# Autodesk Inventor assembly: сборка пульта
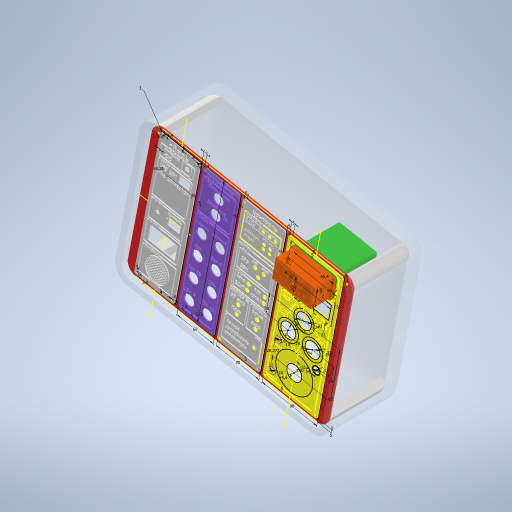
[picture p0: Inventor's stored thumbnail of the model, 512x512]
Saved by Autodesk Inventor 2023.2 (Build 272271000, 271)
## iProperties
Created: 2023-02-13
Part Number: сборка пульта
Document SubType Name: Assembly
Designer: User
Author: User
## Documents named in this file (10)
- C:\Users\matvey\Desktop\YandexDisk\облачное хранилище\НАСУ\Inventor\сборка пульта.iam
- C:\Users\matvey\Desktop\YandexDisk\облачное хранилище\НАСУ\Inventor\Корпус НАСУ.ipt
- C:\Users\matvey\Desktop\YandexDisk\облачное хранилище\НАСУ\Inventor\уголок насу.ipt
- C:\Users\matvey\Desktop\YandexDisk\облачное хранилище\НАСУ\Inventor\рамка насу.ipt
- C:\Users\matvey\Desktop\YandexDisk\облачное хранилище\НАСУ\Inventor\блок пуска.ipt
- C:\Users\matvey\Desktop\YandexDisk\облачное хранилище\НАСУ\Inventor\нижняя часть держателя аккумов.ipt
- C:\Users\matvey\Desktop\YandexDisk\облачное хранилище\НАСУ\Inventor\верхняя часть держателя аккумулятора.ipt
- C:\Users\matvey\Desktop\YandexDisk\облачное хранилище\НАСУ\Inventor\блок управления.ipt
- C:\Users\matvey\Desktop\YandexDisk\облачное хранилище\НАСУ\новый концепт\блок контроля.ipt
- C:\Users\matvey\Desktop\YandexDisk\облачное хранилище\НАСУ\новый концепт\блок антенн.ipt
## Components (12 placed, 9 different names)
1. Корпус НАСУ:1 — Совмещение:1, Вставка:1, Совмещение:2, Угол:1, Совмещение:3, Совмещение:4, Угол:2, Совмещение:5, Совмещение:6, Угол:3, Совмещение:7
2. уголок насу:1 — Совмещение:1, Вставка:1
3. уголок насу:2 — Совмещение:2, Угол:1, Совмещение:3, Совмещение:8, Совмещение:10
4. уголок насу:3 — Совмещение:6, Угол:3, Совмещение:7, Совмещение:9
5. уголок насу:4 — Совмещение:4, Угол:2, Совмещение:5
6. рамка насу:1 — Совмещение:8, Совмещение:9, Совмещение:10, Совмещение:11, Совмещение:12, Совмещение:13, Совмещение:21, Совмещение:22, Совмещение:26, Совмещение:27, Совмещение:28, Совмещение:29, Совмещение:30, Совмещение:31, Совмещение:33
7. нижняя часть держателя аккумов:1 — Совмещение:14, Совмещение:15, Совмещение:16, Совмещение:17, Совмещение:18, Совмещение:32, Совмещение:34
8. верхняя часть держателя аккумулятора:1 — Совмещение:17, Совмещение:18, Совмещение:34
9. блок управления:1 — Совмещение:21, Совмещение:22, Совмещение:33
10. блок контроля:1 — Совмещение:26, Совмещение:27, Совмещение:28
11. блок антенн:1 — Совмещение:29, Совмещение:30, Совмещение:31
12. блок пуска:1 — Совмещение:11, Совмещение:12, Совмещение:13, Совмещение:14, Совмещение:15, Совмещение:16, Совмещение:32
## Relationships (33: Mate 29, Angle 3, Insert 1)
- Совмещение:1 [Mate]: Корпус НАСУ:1 ↔ уголок насу:1
- Вставка:1 [Insert]: Корпус НАСУ:1 ↔ уголок насу:1
- Совмещение:2 [Mate]: Корпус НАСУ:1 ↔ уголок насу:2
- Угол:1 [Angle] (0 deg): Корпус НАСУ:1 ↔ уголок насу:2
- Совмещение:3 [Mate]: Корпус НАСУ:1 ↔ уголок насу:2
- Совмещение:4 [Mate]: Корпус НАСУ:1 ↔ уголок насу:4
- Угол:2 [Angle] (180 deg): Корпус НАСУ:1 ↔ уголок насу:4
- Совмещение:5 [Mate]: Корпус НАСУ:1 ↔ уголок насу:4
- Совмещение:6 [Mate]: Корпус НАСУ:1 ↔ уголок насу:3
- Угол:3 [Angle] (270 deg): Корпус НАСУ:1 ↔ уголок насу:3
- Совмещение:7 [Mate]: Корпус НАСУ:1 ↔ уголок насу:3
- Совмещение:8 [Mate]: уголок насу:2 ↔ рамка насу:1
- Совмещение:9 [Mate]: уголок насу:3 ↔ рамка насу:1
- Совмещение:10 [Mate]: уголок насу:2 ↔ рамка насу:1
- Совмещение:11 [Mate]: рамка насу:1 ↔ блок пуска:1
- Совмещение:12 [Mate]: рамка насу:1 ↔ блок пуска:1
- Совмещение:13 [Mate]: рамка насу:1 ↔ блок пуска:1
- Совмещение:14 [Mate]: нижняя часть держателя аккумов:1 ↔ блок пуска:1
- Совмещение:15 [Mate]: нижняя часть держателя аккумов:1 ↔ блок пуска:1
- Совмещение:16 [Mate]: нижняя часть держателя аккумов:1 ↔ блок пуска:1
- Совмещение:17 [Mate]: нижняя часть держателя аккумов:1 ↔ верхняя часть держателя аккумулятора:1
- Совмещение:18 [Mate]: нижняя часть держателя аккумов:1 ↔ верхняя часть держателя аккумулятора:1
- Совмещение:21 [Mate]: рамка насу:1 ↔ блок управления:1
- Совмещение:22 [Mate]: рамка насу:1 ↔ блок управления:1
- Совмещение:26 [Mate]: рамка насу:1 ↔ блок контроля:1
- Совмещение:27 [Mate]: рамка насу:1 ↔ блок контроля:1
- Совмещение:28 [Mate]: рамка насу:1 ↔ блок контроля:1
- Совмещение:29 [Mate]: рамка насу:1 ↔ блок антенн:1
- Совмещение:30 [Mate]: рамка насу:1 ↔ блок антенн:1
- Совмещение:31 [Mate]: рамка насу:1 ↔ блок антенн:1
- Совмещение:32 [Mate]: нижняя часть держателя аккумов:1 ↔ блок пуска:1
- Совмещение:33 [Mate]: рамка насу:1 ↔ блок управления:1
- Совмещение:34 [Mate]: нижняя часть держателя аккумов:1 ↔ верхняя часть держателя аккумулятора:1
